# Autodesk Inventor assembly: Assembly1492
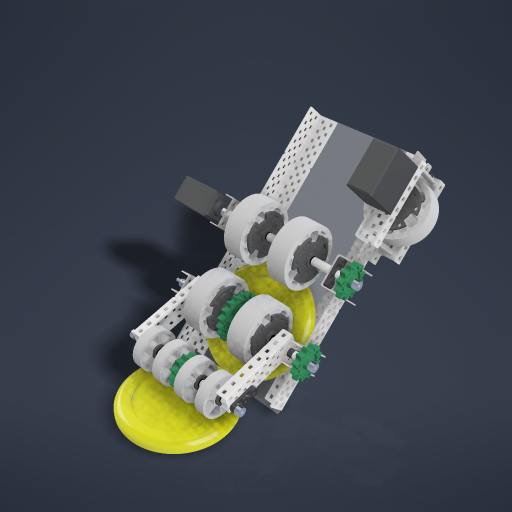
[picture p0: Inventor's stored thumbnail of the model, 512x512]
Saved by Autodesk Inventor 2023 (Build 270158000, 158)
## iProperties
Created: 2023-01-23
Part Number: Assembly1492
Document SubType Name: Assembly
Designer: Windows Macbook
Author: Windows Macbook
## Documents named in this file (45)
- C:\Users\Windows Macbook\Desktop\Inventor\shoot.iam
- C:\Users\Windows Macbook\Documents\Inventor\Content Center Files\VEX-CAD-Inventor-1.4.0\Structure\Plate\Aluminum\Alu Plate 25x25.iam
- C:\Users\Windows Macbook\Documents\Inventor\Content Center Files\VEX-CAD-Inventor-1.4.0\Miscellaneous\Sizing Tool\VRC High School.ipt
- C:\Users\Windows Macbook\Documents\Inventor\Content Center Files\VEX-CAD-Inventor-1.4.0\Miscellaneous\Sizing Tool.ipt
- C:\Users\Windows Macbook\Documents\Inventor\Content Center Files\polycarb10x6.ipt
- C:\Users\Windows Macbook\Documents\Inventor\Content Center Files\276-7500-001 Web.ipt
- C:\Users\Windows Macbook\Documents\Inventor\Content Center Files\VEX-CAD-Inventor-1.4.0\Motion\Wheels\Flex Wheels\2.000 Flex Wheel\2.000 30A .500.ipt
- C:\Users\Windows Macbook\Documents\Inventor\Content Center Files\VEX-CAD-Inventor-1.4.0\Motion\Wheels\Flex Wheels\2.000 Flex Wheel.ipt
- C:\Users\Windows Macbook\Documents\Inventor\Content Center Files\VEX-CAD-Inventor-1.4.0\Motion\Wheels\Flex Wheels\3.000 Flex Wheel\3.000 30A 1.000.ipt
- C:\Users\Windows Macbook\Documents\Inventor\Content Center Files\VEX-CAD-Inventor-1.4.0\Motion\Wheels\Flex Wheels\3.000 Flex Wheel.ipt
- C:\Users\Windows Macbook\Documents\Inventor\Content Center Files\VEX-CAD-Inventor-1.4.0\Structure\C Channel\Aluminum 1x3x1\Alu C 1x3x1x5.ipt
- C:\Users\Windows Macbook\Documents\Inventor\Content Center Files\VEX-CAD-Inventor-1.4.0\Motion\Spacers\Spacer Nylon .313 OD\NSpacer .313 OD x .125.ipt
- C:\Users\Windows Macbook\Documents\Inventor\Content Center Files\VEX-CAD-Inventor-1.4.0\Motion\Spacers\Spacer Nylon .313 OD.ipt
- C:\Users\Windows Macbook\Documents\Inventor\Content Center Files\VEX-CAD-Inventor-1.4.0\Motion\Shaft LS\Shaft Collar Metal.ipt
- C:\Users\Windows Macbook\Documents\Inventor\Content Center Files\VEX-CAD-Inventor-1.4.0\Motion\Wheels\Flex Wheels\VersaHex Adapters .250.ipt
- C:\Users\Windows Macbook\Documents\Inventor\Content Center Files\VEX-CAD-Inventor-1.4.0\Motion\Wheels\Flex Wheels\VersaHub.ipt
- C:\Users\Windows Macbook\Documents\Inventor\Content Center Files\VEX-CAD-Inventor-1.4.0\Motion\Shaft LS\Shaft LS.ipt
- C:\Users\Windows Macbook\Documents\Inventor\Content Center Files\VEX-CAD-Inventor-1.4.0\Motion\Insert Square.ipt
- C:\Users\Windows Macbook\Documents\Inventor\Content Center Files\VEX-CAD-Inventor-1.4.0\Motion\Shaft LS\Bearing Flat.ipt
- C:\Users\Windows Macbook\Documents\Inventor\Content Center Files\VEX-CAD-Inventor-1.4.0\Structure\C Channel\Aluminum 1x2x1\Alu C 1x2x1x8.ipt
- C:\Users\Windows Macbook\Documents\Inventor\Content Center Files\VEX-CAD-Inventor-1.4.0\Motion\Spacers\Spacer Nylon .313 OD\NSpacer .313 OD x .250.ipt
- C:\Users\Windows Macbook\Documents\Inventor\Content Center Files\VEX-CAD-Inventor-1.4.0\Structure\C Channel\Aluminum 1x3x1\Alu C 1x3x1x5_MIR.ipt
- C:\Users\Windows Macbook\Documents\Inventor\Content Center Files\VEX-CAD-Inventor-1.4.0\Motion\Shaft LS\Shaft Collar Metal_MIR2.ipt
- C:\Users\Windows Macbook\Documents\Inventor\Content Center Files\VEX-CAD-Inventor-1.4.0\Motion\Shaft LS\Bearing Flat_MIR2.ipt
- C:\Users\Windows Macbook\Documents\Inventor\Content Center Files\VEX-CAD-Inventor-1.4.0\Structure\C Channel\Aluminum 1x2x1\Alu C 1x2x1x8_MIR2.ipt
- C:\Users\Windows Macbook\Documents\Inventor\Content Center Files\VEX-CAD-Inventor-1.4.0\Motion\Sprockets\9P Sprocket\9P 12T Sprocket, Square.iam
- C:\Users\Windows Macbook\Documents\Inventor\Content Center Files\VEX-CAD-Inventor-1.4.0\Motion\Sprockets\9P Sprocket.iam
- C:\Users\Windows Macbook\Documents\Inventor\Content Center Files\VEX-CAD-Inventor-1.4.0\Motion\Sprockets\9P Sprocket\9P 18T Sprocket, Square.iam
- C:\Users\Windows Macbook\Documents\Inventor\Content Center Files\VEX-CAD-Inventor-1.4.0\Structure\C Channel\Aluminum 1x2x1\Alu C 1x2x1x5.ipt
- C:\Users\Windows Macbook\Documents\Inventor\Content Center Files\VEX-CAD-Inventor-1.4.0\Motion\Spacers\Spacer Nylon .313 OD\NSpacer .313 OD x .500.ipt
- C:\Users\Windows Macbook\Documents\Inventor\Content Center Files\VEX-CAD-Inventor-1.4.0\Motion\Spacers\Spacer Nylon .313 OD\NSpacer .313 OD x .375.ipt
- C:\Users\Windows Macbook\Documents\Inventor\Content Center Files\VEX-CAD-Inventor-1.4.0\Structure\Angle\Aluminum\2x2\Alu Angle 2x2x2.ipt
- C:\Users\Windows Macbook\Documents\Inventor\Content Center Files\VEX-CAD-Inventor-1.4.0\Structure\C Channel\Aluminum 1x2x1\Alu C 1x2x1x10.ipt
- C:\Users\Windows Macbook\Documents\Inventor\Content Center Files\VEX-CAD-Inventor-1.4.0\Structure\Standoff\Standoff 1.50.ipt
- C:\Users\Windows Macbook\Documents\Inventor\Content Center Files\VEX-CAD-Inventor-1.4.0\Structure\Standoff.ipt
- C:\Users\Windows Macbook\Documents\Inventor\Content Center Files\VEX-CAD-Inventor-1.4.0\Motion\Spacers\Washer Teflon.ipt
- C:\Users\Windows Macbook\Documents\Inventor\Content Center Files\VEX-CAD-Inventor-1.4.0\Electronics\V5 Simple Motor.ipt
- C:\Users\Windows Macbook\Documents\Inventor\Content Center Files\VEX-CAD-Inventor-1.4.0\Motion\Shaft LS\Shaft LS\Shaft LS 4.0.ipt
- C:\Users\Windows Macbook\Documents\Inventor\Content Center Files\VEX-CAD-Inventor-1.4.0\Motion\Spacers\Washer Teflon\TWasher .375 OD x .06250.ipt
- C:\Users\Windows Macbook\Documents\Inventor\Content Center Files\VEX-CAD-Inventor-1.4.0\Motion\Spacers\Washer Teflon\TWasher .375 OD x .03125.ipt
- C:\Users\Windows Macbook\Documents\Inventor\Content Center Files\VEX-CAD-Inventor-1.4.0\Motion\Shaft LS\Shaft LS\Shaft LS 8.0.ipt
- C:\Users\Windows Macbook\Documents\Inventor\Content Center Files\VEX-CAD-Inventor-1.4.0\Motion\Shaft LS\Shaft LS\Shaft LS 8.5.ipt
- C:\Users\Windows Macbook\Documents\Inventor\Content Center Files\VEX-CAD-Inventor-1.4.0\Motion\Shaft LS\Shaft LS\Shaft LS 7.0.ipt
- C:\Users\Windows Macbook\Documents\Inventor\Content Center Files\VEX-CAD-Inventor-1.4.0\Structure\Angle\Aluminum\2x2\Alu Angle 2x2x25.ipt
- C:\Users\Windows Macbook\Documents\Inventor\Content Center Files\VEX-CAD-Inventor-1.4.0\Structure\Angle\Aluminum\2x2\Alu Angle 2x2x17.ipt
## Components (137 placed, 36 different names)
1. Alu Plate 25x25:1 [sub-assembly] — Mate:1, Mate:2, Mate:6
2. VRC High School:1 — Mate:1
3. polycarb10x6:1 — Mate:2, Mate:139, Mate:184, Mate:185, Mate:186, Mate:187, Mate:191
4. 276-7500-001 Web:1 — Mate:6
5. 2.000 30A .500:1 — Mate:25, Mate:26, Mate:27, Mate:28, Mate:29, Mate:30, Mate:43
6. 3.000 30A 1.000:2 — Insert:6, Insert:7, Insert:8, Insert:9
7. NSpacer .313 OD x .125:1 — Insert:26, Insert:70
8. VersaHex Adapters .250:1 — Mate:7, Mate:8, Mate:9, Mate:16, Mate:17, Mate:18
9. VersaHub:1 — Mate:16, Mate:17, Mate:18, Insert:6, Insert:7
10. Insert Square:1 — Mate:7, Mate:8, Mate:9, Insert:348
11. VersaHex Adapters .250:2 — Mate:27, Mate:28, Mate:29
12. Insert Square:2 — Insert:83
13. VersaHex Adapters .250:3 — Mate:25, Mate:26, Mate:30, Mate:43
14. Insert Square:3 — Insert:35
15. VersaHex Adapters .250:4
16. VersaHub:2 — Insert:8, Insert:9
17. Insert Square:4 — Insert:424
18. 3.000 30A 1.000:3
19. VersaHex Adapters .250:5
20. VersaHub:3
21. Insert Square:5 — Insert:67
22. VersaHex Adapters .250:6
23. VersaHub:4
24. Insert Square:6 — Mate:142
25. Bearing Flat:1 — Insert:71, Insert:72, Insert:355
26. Bearing Flat:2 — Insert:19, Insert:24, Insert:25
27. Shaft Collar Metal:2 — Insert:19, Flush:19, Cylindrical:14
28. Alu C 1x3x1x5:2 — Insert:31, Insert:32, Insert:101, Insert:425, Insert:426
29. Alu C 1x2x1x8:1 — Insert:24, Insert:25, Insert:26, Insert:34, Insert:88
30. Bearing Flat:3 — Insert:31, Insert:32, Insert:362
31. NSpacer .313 OD x .250:2 — Insert:33, Insert:34
32. NSpacer .313 OD x .250:3 — Insert:33, Insert:35
33. NSpacer .313 OD x .125:4 — Insert:45, Insert:76
34. Bearing Flat_MIR2:1 — Insert:77, Insert:78, Insert:357
35. Bearing Flat_MIR2:2 — Insert:46, Insert:47, Insert:359
36. Alu C 1x3x1x5_MIR:2 — Insert:97, Insert:226, Insert:227, Insert:346, Insert:429, Insert:430
37. Alu C 1x2x1x8_MIR2:1 — Insert:45, Insert:46, Insert:47, Insert:51, Insert:86
38. NSpacer .313 OD x .250:5 — Insert:51, Insert:52
39. NSpacer .313 OD x .250:6 — Insert:52, Insert:53
40. 2.000 30A .500:2
41. VersaHex Adapters .250:7
42. Insert Square:7 — Mate:141, Insert:433
43. VersaHex Adapters .250:8
44. Insert Square:8 — Insert:354
45. 2.000 30A .500:4
46. VersaHex Adapters .250:11
47. Insert Square:11 — Insert:53
48. VersaHex Adapters .250:12
49. Insert Square:12 — Insert:82
50. 2.000 30A .500:5
51. VersaHex Adapters .250:13
52. Insert Square:13 — Insert:353
53. VersaHex Adapters .250:14
54. Insert Square:14 — Mate:140, Insert:434
55. 3.000 30A 1.000:4
56. VersaHex Adapters .250:15
57. VersaHub:5
58. Insert Square:15 — Insert:102
59. VersaHex Adapters .250:16
60. VersaHub:6
61. Insert Square:16 — Insert:349
62. Shaft Collar Metal_MIR2:4 — Insert:357, Flush:18, Cylindrical:13
63. Shaft Collar Metal_MIR2:5 — Insert:359, Cylindrical:16
64. 3.000 30A 1.000:5
65. VersaHex Adapters .250:17
66. VersaHub:7
67. Insert Square:17
68. VersaHex Adapters .250:18
69. VersaHub:8
70. Insert Square:18 — Insert:66
71. 9P 18T Sprocket, Square:3 [sub-assembly] — Insert:68, Insert:69
72. NSpacer .313 OD x .250:7 — Insert:67, Insert:69, Insert:223
73. NSpacer .313 OD x .250:8 — Insert:66, Insert:68, Insert:224
74. 276-7500-001 Web:2 — Mate:139
75. Alu C 1x2x1x5:1 — Insert:70, Insert:71, Insert:72, Insert:427, Insert:428
76. Alu C 1x2x1x5:2 — Insert:76, Insert:77, Insert:78, Insert:431, Insert:432
77. NSpacer .313 OD x .500:9 — Insert:83, Mate:140, Insert:434
78. NSpacer .313 OD x .500:10 — Insert:82, Mate:141, Insert:433
79. NSpacer .313 OD x .375:12 — Insert:85, Insert:86
80. NSpacer .313 OD x .375:13 — Insert:85
81. NSpacer .313 OD x .375:14 — Insert:87, Insert:88
82. NSpacer .313 OD x .375:15 — Insert:87, Mate:142
83. NSpacer .313 OD x .375:18 — Insert:93, Insert:97
84. NSpacer .313 OD x .375:19 — Insert:93, Insert:99
85. NSpacer .313 OD x .375:21 — Insert:101
86. NSpacer .313 OD x .375:22 — Insert:100
87. NSpacer .313 OD x .250:24 — Insert:99, Insert:102
88. NSpacer .313 OD x .250:25 — Insert:100, Insert:424
89. 3.000 30A 1.000:7
90. VersaHex Adapters .250:19
91. VersaHub:9
92. Insert Square:19 — Insert:395
93. VersaHex Adapters .250:20
94. VersaHub:10
95. Insert Square:20 — Mate:188, Mate:190, Insert:393
96. Standoff 1.50:2 — Insert:400, Insert:401
97. V5 Simple Motor:1
98. Shaft LS 4.0:4 — Flush:8, Cylindrical:7, Mate:188, Mate:190
99. Bearing Flat:4 — Insert:210
100. Shaft Collar Metal:4 — Insert:210, Flush:8, Cylindrical:7
101. Shaft Collar Metal:5
102. TWasher .375 OD x .06250:9 — Insert:224
103. TWasher .375 OD x .06250:10 — Insert:223
104. V5 Simple Motor:2 — Insert:226, Insert:227
105. NSpacer .313 OD x .250:33 — Insert:417, Insert:418
106. Shaft Collar Metal:7 — Insert:346
107. Shaft LS 8.5:8 — Flush:18, Cylindrical:13
108. NSpacer .313 OD x .500:43 — Insert:348
109. NSpacer .313 OD x .500:44 — Insert:349, Insert:350
110. NSpacer .313 OD x .125:45 — Insert:350
111. 9P 12T Sprocket, Square:4 [sub-assembly] — Insert:352
112. TWasher .375 OD x .03125:17 — Insert:352, Insert:353
113. TWasher .375 OD x .03125:18 — Insert:354
114. 9P 12T Sprocket, Square:5 [sub-assembly] — Insert:356, Insert:358
115. NSpacer .313 OD x .375:47 — Insert:355, Insert:356
116. Shaft Collar Metal:9 — Insert:358
117. Shaft LS 7.0:10 — Flush:19, Cylindrical:14, Cylindrical:16
118. 9P 12T Sprocket, Square:6 [sub-assembly] — Insert:363
119. Shaft Collar Metal:10 — Flush:20, Cylindrical:15
120. NSpacer .313 OD x .375:48 — Insert:362, Insert:363
121. Shaft LS 8.0:11 — Flush:20, Cylindrical:15
122. Standoff 1.50:5 — Insert:397, Insert:398
123. NSpacer .313 OD x .250:49 — Insert:391, Insert:415
124. NSpacer .313 OD x .250:50 — Insert:390, Insert:414
125. NSpacer .313 OD x .250:51 — Insert:416, Insert:419
126. Alu Angle 2x2x25:2 — Mate:184, Mate:185, Flush:21, Mate:191, Insert:429, Insert:430, Insert:431, Insert:432
127. Alu Angle 2x2x17:1 — Mate:186, Mate:187, Flush:21, Insert:390, Insert:391, Insert:425, Insert:426, Insert:427, Insert:428
128. NSpacer .313 OD x .125:52 — Insert:393
129. NSpacer .313 OD x .125:53 — Insert:395
130. NSpacer .313 OD x .125:54 — Insert:401, Insert:421
131. NSpacer .313 OD x .125:55 — Insert:397, Insert:420
132. NSpacer .313 OD x .125:56 — Insert:400, Insert:423
133. NSpacer .313 OD x .125:57 — Insert:398, Insert:422
134. Alu Angle 2x2x2:1 — Insert:418, Insert:419
135. Alu C 1x2x1x8:2 — Insert:420, Insert:421
136. Alu C 1x2x1x8:3 — Insert:412, Insert:413, Insert:422, Insert:423
137. Alu C 1x2x1x10:4 — Insert:412, Insert:413, Insert:414, Insert:415, Insert:416, Insert:417
## Relationships (245: Mate 126, Insert 109, Flush 5, CylindricalJoint 5)
- Mate:1: Alu Plate 25x25:1 ↔ VRC High School:1
- Mate:2: Alu Plate 25x25:1 ↔ polycarb10x6:1
- Mate:6: Alu Plate 25x25:1 ↔ 276-7500-001 Web:1
- Mate:7: VersaHex Adapters .250:1 ↔ Insert Square:1
- Mate:8: VersaHex Adapters .250:1 ↔ Insert Square:1
- Mate:9: VersaHex Adapters .250:1 ↔ Insert Square:1
- [Mate]: VersaHex Adapters .250:2 ↔ Insert Square:2
- [Mate]: VersaHex Adapters .250:2 ↔ Insert Square:2
- [Mate]: VersaHex Adapters .250:2 ↔ Insert Square:2
- [Mate]: VersaHex Adapters .250:3 ↔ Insert Square:3
- [Mate]: VersaHex Adapters .250:3 ↔ Insert Square:3
- [Mate]: VersaHex Adapters .250:3 ↔ Insert Square:3
- Mate:16: VersaHex Adapters .250:1 ↔ VersaHub:1
- Mate:17: VersaHex Adapters .250:1 ↔ VersaHub:1
- Mate:18: VersaHex Adapters .250:1 ↔ VersaHub:1
- [Mate]: VersaHex Adapters .250:4 ↔ Insert Square:4
- [Mate]: VersaHex Adapters .250:4 ↔ Insert Square:4
- [Mate]: VersaHex Adapters .250:4 ↔ Insert Square:4
- [Mate]: VersaHex Adapters .250:4 ↔ VersaHub:2
- [Mate]: VersaHex Adapters .250:4 ↔ VersaHub:2
- [Mate]: VersaHex Adapters .250:4 ↔ VersaHub:2
- Insert:6: 3.000 30A 1.000:2 ↔ VersaHub:1
- Insert:7: 3.000 30A 1.000:2 ↔ VersaHub:1
- Insert:8: 3.000 30A 1.000:2 ↔ VersaHub:2
- Insert:9: 3.000 30A 1.000:2 ↔ VersaHub:2
- Mate:25 (-1.6002 mm): 2.000 30A .500:1 ↔ VersaHex Adapters .250:3
- Mate:26 (-1.6002 mm): 2.000 30A .500:1 ↔ VersaHex Adapters .250:3
- Mate:27 (-1.6002 mm): 2.000 30A .500:1 ↔ VersaHex Adapters .250:2
- Mate:28 (-1.6002 mm): 2.000 30A .500:1 ↔ VersaHex Adapters .250:2
- Mate:29: 2.000 30A .500:1 ↔ VersaHex Adapters .250:2
- Mate:30: 2.000 30A .500:1 ↔ VersaHex Adapters .250:3
- [Mate]: VersaHex Adapters .250:5 ↔ Insert Square:5
- [Mate]: VersaHex Adapters .250:5 ↔ Insert Square:5
- [Mate]: VersaHex Adapters .250:5 ↔ Insert Square:5
- [Mate]: VersaHex Adapters .250:5 ↔ VersaHub:3
- [Mate]: VersaHex Adapters .250:5 ↔ VersaHub:3
- [Mate]: VersaHex Adapters .250:5 ↔ VersaHub:3
- [Mate]: VersaHex Adapters .250:6 ↔ Insert Square:6
- [Mate]: VersaHex Adapters .250:6 ↔ Insert Square:6
- [Mate]: VersaHex Adapters .250:6 ↔ Insert Square:6
- [Mate]: VersaHex Adapters .250:6 ↔ VersaHub:4
- [Mate]: VersaHex Adapters .250:6 ↔ VersaHub:4
- [Mate]: VersaHex Adapters .250:6 ↔ VersaHub:4
- [Insert]: 3.000 30A 1.000:3 ↔ VersaHub:3
- [Insert]: 3.000 30A 1.000:3 ↔ VersaHub:3
- [Insert]: 3.000 30A 1.000:3 ↔ VersaHub:4
- [Insert]: 3.000 30A 1.000:3 ↔ VersaHub:4
- Insert:19: Bearing Flat:2 ↔ Shaft Collar Metal:2
- Mate:43: 2.000 30A .500:1 ↔ VersaHex Adapters .250:3
- Insert:24: Bearing Flat:2 ↔ Alu C 1x2x1x8:1
- Insert:25: Bearing Flat:2 ↔ Alu C 1x2x1x8:1
- Insert:26: NSpacer .313 OD x .125:1 ↔ Alu C 1x2x1x8:1
- Insert:31: Alu C 1x3x1x5:2 ↔ Bearing Flat:3
- Insert:32: Alu C 1x3x1x5:2 ↔ Bearing Flat:3
- Insert:33: NSpacer .313 OD x .250:2 ↔ NSpacer .313 OD x .250:3
- Insert:34: Alu C 1x2x1x8:1 ↔ NSpacer .313 OD x .250:2
- Insert:35: Insert Square:3 ↔ NSpacer .313 OD x .250:3
- Insert:45: NSpacer .313 OD x .125:4 ↔ Alu C 1x2x1x8_MIR2:1
- Insert:46: Bearing Flat_MIR2:2 ↔ Alu C 1x2x1x8_MIR2:1
- Insert:47: Bearing Flat_MIR2:2 ↔ Alu C 1x2x1x8_MIR2:1
- Insert:51: Alu C 1x2x1x8_MIR2:1 ↔ NSpacer .313 OD x .250:5
- Insert:52: NSpacer .313 OD x .250:5 ↔ NSpacer .313 OD x .250:6
- [Mate]: VersaHex Adapters .250:7 ↔ Insert Square:7
- [Mate]: VersaHex Adapters .250:7 ↔ Insert Square:7
- [Mate]: VersaHex Adapters .250:7 ↔ Insert Square:7
- [Mate]: VersaHex Adapters .250:8 ↔ Insert Square:8
- [Mate]: VersaHex Adapters .250:8 ↔ Insert Square:8
- [Mate]: VersaHex Adapters .250:8 ↔ Insert Square:8
- [Mate] (-1.6002 mm): 2.000 30A .500:2 ↔ VersaHex Adapters .250:8
- [Mate] (-1.6002 mm): 2.000 30A .500:2 ↔ VersaHex Adapters .250:8
- [Mate] (-1.6002 mm): 2.000 30A .500:2 ↔ VersaHex Adapters .250:7
- [Mate] (-1.6002 mm): 2.000 30A .500:2 ↔ VersaHex Adapters .250:7
- [Mate]: 2.000 30A .500:2 ↔ VersaHex Adapters .250:7
- [Mate]: 2.000 30A .500:2 ↔ VersaHex Adapters .250:8
- [Mate]: 2.000 30A .500:2 ↔ VersaHex Adapters .250:8
- [Mate]: VersaHex Adapters .250:11 ↔ Insert Square:11
- [Mate]: VersaHex Adapters .250:11 ↔ Insert Square:11
- [Mate]: VersaHex Adapters .250:11 ↔ Insert Square:11
- [Mate]: VersaHex Adapters .250:12 ↔ Insert Square:12
- [Mate]: VersaHex Adapters .250:12 ↔ Insert Square:12
- [Mate]: VersaHex Adapters .250:12 ↔ Insert Square:12
- [Mate] (-1.6002 mm): 2.000 30A .500:4 ↔ VersaHex Adapters .250:12
- [Mate] (-1.6002 mm): 2.000 30A .500:4 ↔ VersaHex Adapters .250:12
- [Mate] (-1.6002 mm): 2.000 30A .500:4 ↔ VersaHex Adapters .250:11
- [Mate] (-1.6002 mm): 2.000 30A .500:4 ↔ VersaHex Adapters .250:11
- [Mate]: 2.000 30A .500:4 ↔ VersaHex Adapters .250:11
- [Mate]: 2.000 30A .500:4 ↔ VersaHex Adapters .250:12
- [Mate]: 2.000 30A .500:4 ↔ VersaHex Adapters .250:12
- [Mate]: VersaHex Adapters .250:13 ↔ Insert Square:13
- [Mate]: VersaHex Adapters .250:13 ↔ Insert Square:13
- [Mate]: VersaHex Adapters .250:13 ↔ Insert Square:13
- [Mate]: VersaHex Adapters .250:14 ↔ Insert Square:14
- [Mate]: VersaHex Adapters .250:14 ↔ Insert Square:14
- [Mate]: VersaHex Adapters .250:14 ↔ Insert Square:14
- [Mate] (-1.6002 mm): 2.000 30A .500:5 ↔ VersaHex Adapters .250:14
- [Mate] (-1.6002 mm): 2.000 30A .500:5 ↔ VersaHex Adapters .250:14
- [Mate] (-1.6002 mm): 2.000 30A .500:5 ↔ VersaHex Adapters .250:13
- [Mate] (-1.6002 mm): 2.000 30A .500:5 ↔ VersaHex Adapters .250:13
- [Mate]: 2.000 30A .500:5 ↔ VersaHex Adapters .250:13
- [Mate]: 2.000 30A .500:5 ↔ VersaHex Adapters .250:14
- [Mate]: 2.000 30A .500:5 ↔ VersaHex Adapters .250:14
- Insert:53: NSpacer .313 OD x .250:6 ↔ Insert Square:11
- [Mate]: VersaHex Adapters .250:15 ↔ Insert Square:15
- [Mate]: VersaHex Adapters .250:15 ↔ Insert Square:15
- [Mate]: VersaHex Adapters .250:15 ↔ Insert Square:15
- [Mate]: VersaHex Adapters .250:15 ↔ VersaHub:5
- [Mate]: VersaHex Adapters .250:15 ↔ VersaHub:5
- [Mate]: VersaHex Adapters .250:15 ↔ VersaHub:5
- [Mate]: VersaHex Adapters .250:16 ↔ Insert Square:16
- [Mate]: VersaHex Adapters .250:16 ↔ Insert Square:16
- [Mate]: VersaHex Adapters .250:16 ↔ Insert Square:16
- [Mate]: VersaHex Adapters .250:16 ↔ VersaHub:6
- [Mate]: VersaHex Adapters .250:16 ↔ VersaHub:6
- [Mate]: VersaHex Adapters .250:16 ↔ VersaHub:6
- [Insert]: 3.000 30A 1.000:4 ↔ VersaHub:5
- [Insert]: 3.000 30A 1.000:4 ↔ VersaHub:5
- [Insert]: 3.000 30A 1.000:4 ↔ VersaHub:6
- [Insert]: 3.000 30A 1.000:4 ↔ VersaHub:6
- [Mate]: VersaHex Adapters .250:17 ↔ Insert Square:17
- [Mate]: VersaHex Adapters .250:17 ↔ Insert Square:17
- [Mate]: VersaHex Adapters .250:17 ↔ Insert Square:17
- [Mate]: VersaHex Adapters .250:17 ↔ VersaHub:7
- [Mate]: VersaHex Adapters .250:17 ↔ VersaHub:7
- [Mate]: VersaHex Adapters .250:17 ↔ VersaHub:7
- [Mate]: VersaHex Adapters .250:18 ↔ Insert Square:18
- [Mate]: VersaHex Adapters .250:18 ↔ Insert Square:18
- [Mate]: VersaHex Adapters .250:18 ↔ Insert Square:18
- [Mate]: VersaHex Adapters .250:18 ↔ VersaHub:8
- [Mate]: VersaHex Adapters .250:18 ↔ VersaHub:8
- [Mate]: VersaHex Adapters .250:18 ↔ VersaHub:8
- [Insert]: 3.000 30A 1.000:5 ↔ VersaHub:7
- [Insert]: 3.000 30A 1.000:5 ↔ VersaHub:7
- [Insert]: 3.000 30A 1.000:5 ↔ VersaHub:8
- [Insert]: 3.000 30A 1.000:5 ↔ VersaHub:8
- Insert:66: Insert Square:18 ↔ NSpacer .313 OD x .250:8
- Insert:67: Insert Square:5 ↔ NSpacer .313 OD x .250:7
- Insert:68 (1.9304 mm): 9P 18T Sprocket, Square:3 ↔ NSpacer .313 OD x .250:8
- Insert:69 (1.9304 mm): 9P 18T Sprocket, Square:3 ↔ NSpacer .313 OD x .250:7
- Mate:139: polycarb10x6:1 ↔ 276-7500-001 Web:2
- Insert:70: NSpacer .313 OD x .125:1 ↔ Alu C 1x2x1x5:1
- Insert:71: Bearing Flat:1 ↔ Alu C 1x2x1x5:1
- Insert:72: Bearing Flat:1 ↔ Alu C 1x2x1x5:1
- Insert:76: NSpacer .313 OD x .125:4 ↔ Alu C 1x2x1x5:2
- Insert:77: Bearing Flat_MIR2:1 ↔ Alu C 1x2x1x5:2
- Insert:78: Bearing Flat_MIR2:1 ↔ Alu C 1x2x1x5:2
- Insert:82: Insert Square:12 ↔ NSpacer .313 OD x .500:10
- Insert:83: Insert Square:2 ↔ NSpacer .313 OD x .500:9
- Mate:140: Insert Square:14 ↔ NSpacer .313 OD x .500:9
- Mate:141: Insert Square:7 ↔ NSpacer .313 OD x .500:10
- Insert:85: NSpacer .313 OD x .375:12 ↔ NSpacer .313 OD x .375:13
- Insert:86: Alu C 1x2x1x8_MIR2:1 ↔ NSpacer .313 OD x .375:12
- Insert:87: NSpacer .313 OD x .375:14 ↔ NSpacer .313 OD x .375:15
- Insert:88: Alu C 1x2x1x8:1 ↔ NSpacer .313 OD x .375:14
- Mate:142: Insert Square:6 ↔ NSpacer .313 OD x .375:15
- Insert:93: NSpacer .313 OD x .375:18 ↔ NSpacer .313 OD x .375:19
- [Insert]: NSpacer .313 OD x .375:21 ↔ NSpacer .313 OD x .375:22
- Insert:97: Alu C 1x3x1x5_MIR:2 ↔ NSpacer .313 OD x .375:18
- Insert:99: NSpacer .313 OD x .375:19 ↔ NSpacer .313 OD x .250:24
- Insert:100: NSpacer .313 OD x .375:22 ↔ NSpacer .313 OD x .250:25
- Insert:101: Alu C 1x3x1x5:2 ↔ NSpacer .313 OD x .375:21
- Insert:102: Insert Square:15 ↔ NSpacer .313 OD x .250:24
- [Mate]: VersaHex Adapters .250:19 ↔ Insert Square:19
- [Mate]: VersaHex Adapters .250:19 ↔ Insert Square:19
- [Mate]: VersaHex Adapters .250:19 ↔ Insert Square:19
- [Mate]: VersaHex Adapters .250:19 ↔ VersaHub:9
- [Mate]: VersaHex Adapters .250:19 ↔ VersaHub:9
- [Mate]: VersaHex Adapters .250:19 ↔ VersaHub:9
- [Mate]: VersaHex Adapters .250:20 ↔ Insert Square:20
- [Mate]: VersaHex Adapters .250:20 ↔ Insert Square:20
- [Mate]: VersaHex Adapters .250:20 ↔ Insert Square:20
- [Mate]: VersaHex Adapters .250:20 ↔ VersaHub:10
- [Mate]: VersaHex Adapters .250:20 ↔ VersaHub:10
- [Mate]: VersaHex Adapters .250:20 ↔ VersaHub:10
- [Insert]: 3.000 30A 1.000:7 ↔ VersaHub:9
- [Insert]: 3.000 30A 1.000:7 ↔ VersaHub:9
- [Insert]: 3.000 30A 1.000:7 ↔ VersaHub:10
- [Insert]: 3.000 30A 1.000:7 ↔ VersaHub:10
- Insert:210: Bearing Flat:4 ↔ Shaft Collar Metal:4
- Flush:8: Shaft LS 4.0:4 ↔ Shaft Collar Metal:4
- Cylindrical:7: Shaft LS 4.0:4 ↔ Shaft Collar Metal:4
- Insert:223: NSpacer .313 OD x .250:7 ↔ TWasher .375 OD x .06250:10
- Insert:224: NSpacer .313 OD x .250:8 ↔ TWasher .375 OD x .06250:9
- Insert:226: Alu C 1x3x1x5_MIR:2 ↔ V5 Simple Motor:2
- Insert:227: Alu C 1x3x1x5_MIR:2 ↔ V5 Simple Motor:2
- Insert:346: Alu C 1x3x1x5_MIR:2 ↔ Shaft Collar Metal:7
- Insert:348: Insert Square:1 ↔ NSpacer .313 OD x .500:43
- Insert:349: Insert Square:16 ↔ NSpacer .313 OD x .500:44
- Insert:350: NSpacer .313 OD x .500:44 ↔ NSpacer .313 OD x .125:45
- Insert:352: 9P 12T Sprocket, Square:4 ↔ TWasher .375 OD x .03125:17
- Insert:353: Insert Square:13 ↔ TWasher .375 OD x .03125:17
- Insert:354: Insert Square:8 ↔ TWasher .375 OD x .03125:18
- Insert:355: Bearing Flat:1 ↔ NSpacer .313 OD x .375:47
- Insert:356: 9P 12T Sprocket, Square:5 ↔ NSpacer .313 OD x .375:47
- Insert:357: Bearing Flat_MIR2:1 ↔ Shaft Collar Metal_MIR2:4
- Flush:18 (-8.89 mm): Shaft Collar Metal_MIR2:4 ↔ Shaft LS 8.5:8
- Cylindrical:13: Shaft Collar Metal_MIR2:4 ↔ Shaft LS 8.5:8
- Insert:358: 9P 12T Sprocket, Square:5 ↔ Shaft Collar Metal:9
- Insert:359: Bearing Flat_MIR2:2 ↔ Shaft Collar Metal_MIR2:5
- Flush:19: Shaft Collar Metal:2 ↔ Shaft LS 7.0:10
- Cylindrical:14: Shaft Collar Metal:2 ↔ Shaft LS 7.0:10
- [Insert]: 9P 12T Sprocket, Square:6 ↔ Shaft Collar Metal:10
- Insert:362: Bearing Flat:3 ↔ NSpacer .313 OD x .375:48
- Insert:363: 9P 12T Sprocket, Square:6 ↔ NSpacer .313 OD x .375:48
- Flush:20: Shaft Collar Metal:10 ↔ Shaft LS 8.0:11
- Cylindrical:15: Shaft Collar Metal:10 ↔ Shaft LS 8.0:11
- Mate:184: polycarb10x6:1 ↔ Alu Angle 2x2x25:2
- Mate:185: polycarb10x6:1 ↔ Alu Angle 2x2x25:2
- Mate:186: polycarb10x6:1 ↔ Alu Angle 2x2x17:1
- Mate:187: polycarb10x6:1 ↔ Alu Angle 2x2x17:1
- Flush:21: Alu Angle 2x2x25:2 ↔ Alu Angle 2x2x17:1
- Insert:390: NSpacer .313 OD x .250:50 ↔ Alu Angle 2x2x17:1
- Insert:391: NSpacer .313 OD x .250:49 ↔ Alu Angle 2x2x17:1
- Mate:188: Insert Square:20 ↔ Shaft LS 4.0:4
- Mate:190: Insert Square:20 ↔ Shaft LS 4.0:4
- Insert:393: Insert Square:20 ↔ NSpacer .313 OD x .125:52
- Insert:395: Insert Square:19 ↔ NSpacer .313 OD x .125:53
- Insert:397: Standoff 1.50:5 ↔ NSpacer .313 OD x .125:55
- Insert:398: Standoff 1.50:5 ↔ NSpacer .313 OD x .125:57
- Insert:400: Standoff 1.50:2 ↔ NSpacer .313 OD x .125:56
- Insert:401: Standoff 1.50:2 ↔ NSpacer .313 OD x .125:54
- Mate:191: polycarb10x6:1 ↔ Alu Angle 2x2x25:2
- Insert:412: Alu C 1x2x1x8:3 ↔ Alu C 1x2x1x10:4
- Insert:413: Alu C 1x2x1x8:3 ↔ Alu C 1x2x1x10:4
- Insert:414: NSpacer .313 OD x .250:50 ↔ Alu C 1x2x1x10:4
- Insert:415: NSpacer .313 OD x .250:49 ↔ Alu C 1x2x1x10:4
- Insert:416: NSpacer .313 OD x .250:51 ↔ Alu C 1x2x1x10:4
- Insert:417: NSpacer .313 OD x .250:33 ↔ Alu C 1x2x1x10:4
- Insert:418: NSpacer .313 OD x .250:33 ↔ Alu Angle 2x2x2:1
- Insert:419: NSpacer .313 OD x .250:51 ↔ Alu Angle 2x2x2:1
- Insert:420: NSpacer .313 OD x .125:55 ↔ Alu C 1x2x1x8:2
- Insert:421: NSpacer .313 OD x .125:54 ↔ Alu C 1x2x1x8:2
- Insert:422: NSpacer .313 OD x .125:57 ↔ Alu C 1x2x1x8:3
- Insert:423: NSpacer .313 OD x .125:56 ↔ Alu C 1x2x1x8:3
- Insert:424: Insert Square:4 ↔ NSpacer .313 OD x .250:25
- Insert:425: Alu C 1x3x1x5:2 ↔ Alu Angle 2x2x17:1
- Insert:426: Alu C 1x3x1x5:2 ↔ Alu Angle 2x2x17:1
- Insert:427: Alu C 1x2x1x5:1 ↔ Alu Angle 2x2x17:1
- Insert:428: Alu C 1x2x1x5:1 ↔ Alu Angle 2x2x17:1
- Insert:429: Alu C 1x3x1x5_MIR:2 ↔ Alu Angle 2x2x25:2
- Insert:430: Alu C 1x3x1x5_MIR:2 ↔ Alu Angle 2x2x25:2
- Insert:431: Alu C 1x2x1x5:2 ↔ Alu Angle 2x2x25:2
- Insert:432: Alu C 1x2x1x5:2 ↔ Alu Angle 2x2x25:2
- Cylindrical:16: Shaft Collar Metal_MIR2:5 ↔ Shaft LS 7.0:10
- Insert:433: Insert Square:7 ↔ NSpacer .313 OD x .500:10
- Insert:434: Insert Square:14 ↔ NSpacer .313 OD x .500:9
## Named parameters: d14_d11 = 0 mm, d15_d12 = 0 mm, d16_d13 = 0 mm, d17_d11 = 0 mm, d18_d12 = 0 mm, d19_d13 = 0 mm, d23_d11 = 0 mm, d24_d12 = 0 mm, d25_d13 = 0 mm, d26_d20 = 0 mm, d27_d21 = 0 mm, d28_d22 = 0 mm, d42_d11 = 0 mm, d43_d12 = 0 mm, d44_d13 = 0 mm, d45_d20 = 0 mm, d46_d21 = 0 mm, d47_d22 = 0 mm, d48_d23_d11 = 0 mm, d49_d24_d12 = 0 mm, d50_d25_d13 = 0 mm, d51_d26_d20 = 0 mm, d52_d27_d21 = 0 mm, d53_d28_d22 = 0 mm, d54_d29 = 0 mm, d55_d30 = 0 mm, d56_d31 = 0 mm, d57_d32 = 0 mm, d126_d70 = 0 mm, d127_d14_d11 = 0 mm, d128_d15_d12 = 0 mm, d129_d16_d13 = 0 mm, d130_d17_d11 = 0 mm, d131_d18_d12 = 0 mm, d132_d19_d13 = 0 mm, d133_d36 = -1.6002 mm, d134_d37 = -1.6002 mm, d135_d38 = -1.6002 mm, d136_d39 = -1.6002 mm, d137_d40 = 0 mm, d138_d41 = 0 mm, d152_d70 = 0 mm, d153_d14_d11 = 0 mm, d154_d15_d12 = 0 mm, d155_d16_d13 = 0 mm, d156_d17_d11 = 0 mm, d157_d18_d12 = 0 mm, d158_d19_d13 = 0 mm, d159_d36 = -1.6002 mm, d160_d37 = -1.6002 mm, d161_d38 = -1.6002 mm, d162_d39 = -1.6002 mm, d163_d40 = 0 mm, d164_d41 = 0 mm, d170_d70 = 0 mm, d171_d14_d11 = 0 mm, d172_d15_d12 = 0 mm, d173_d16_d13 = 0 mm, d174_d17_d11 = 0 mm, d175_d18_d12 = 0 mm, d176_d19_d13 = 0 mm, d177_d36 = -1.6002 mm, d178_d37 = -1.6002 mm, d179_d38 = -1.6002 mm, d180_d39 = -1.6002 mm, d181_d40 = 0 mm, d182_d41 = 0 mm, d186_d42_d11 = 0 mm, d187_d43_d12 = 0 mm, d188_d44_d13 = 0 mm, d189_d45_d20 = 0 mm, d190_d46_d21 = 0 mm, d191_d47_d22 = 0 mm, d192_d48_d23_d11 = 0 mm, d193_d49_d24_d12 = 0 mm, d194_d50_d25_d13 = 0 mm, d195_d51_d26_d20 = 0 mm, d196_d52_d27_d21 = 0 mm, d197_d53_d28_d22 = 0 mm, d198_d54_d29 = 0 mm, d199_d55_d30 = 0 mm, d200_d56_d31 = 0 mm, d201_d57_d32 = 0 mm, d206_d186_d42_d11 = 0 mm, d207_d187_d43_d12 = 0 mm, d208_d188_d44_d13 = 0 mm, d209_d189_d45_d20 = 0 mm, d210_d190_d46_d21 = 0 mm, d211_d191_d47_d22 = 0 mm, d212_d192_d48_d23_d11 = 0 mm, d213_d193_d49_d24_d12 = 0 mm, d214_d194_d50_d25_d13 = 0 mm, d215_d195_d51_d26_d20 = 0 mm, d216_d196_d52_d27_d21 = 0 mm, d217_d197_d53_d28_d22 = 0 mm, d218_d198_d54_d29 = 0 mm, d219_d199_d55_d30 = 0 mm, d220_d200_d56_d31 = 0 mm, d221_d201_d57_d32 = 0 mm, d259_d257 = 0 mm, d392_d11 = 0 mm, d393_d12 = 0 mm, d394_d13 = 0 mm, d395_d20 = 0 mm, d396_d21 = 0 mm, d397_d22 = 0 mm, d398_d23_d11 = 0 mm, d399_d24_d12 = 0 mm, d400_d25_d13 = 0 mm, d401_d26_d20 = 0 mm, d402_d27_d21 = 0 mm, d403_d28_d22 = 0 mm, d404_d29 = 0 mm, d405_d30 = 0 mm, d406_d31 = 0 mm, d407_d32 = 0 mm, d700_d694 = 0 mm
